# Autodesk Inventor assembly: Hoja oculta
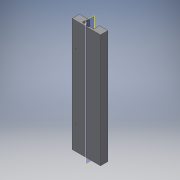
[picture p0: Inventor's stored thumbnail of the model, 180x180]
Saved by Autodesk Inventor 2016 (Build 200138000, 138)
## iProperties
Created: 2015-08-31
Part Number: Hoja oculta
Document SubType Name: Assembly
Designer: amatiasq
Author: amatiasq
## Documents named in this file (4)
- C:\Users\amatiasq\Documents\GitHub\3D\Hoja Oculta\Hoja oculta.iam
- C:\Users\amatiasq\Documents\GitHub\3D\Hoja Oculta\Base.ipt
- C:\Users\amatiasq\Documents\GitHub\3D\Hoja Oculta\Hoja.ipt
- C:\Users\amatiasq\Documents\GitHub\3D\Hoja Oculta\Parametros.xlsx
## Components (2 placed, 2 different names)
1. Base:1 — Mate:1, Flush:1
2. Hoja:1 — Mate:1, Mate:2
## Relationships (3: Mate 2, Flush 1)
- Mate:1 (0.3 mm): Base:1 ↔ Hoja:1
- Flush:1 (-25 mm): Base:1
- Mate:2: Hoja:1
## Named parameters: margen = 0.3 mm, base_largo = 200 mm, base_ancho = 50 mm, base_alto = 3 mm, muros_grosor = 3 mm, muros_alto = 10 mm, rail_alto = 1.5 mm, rail_grosor = 5 mm, hoja_ancho = 20 mm, hoja_largo = 200 mm, hoja_filo = 100 mm, hoja_stop_posicion = 5 mm, hoja_stop_saliente = 5 mm, hoja_stop_largo = 5 mm, hoja_alto = 3 mm, hoja_stop_biselado = 2 mm, hoja_filo_biselado = 0.5 mm, hoja_cola_biselado = 1 mm
